# Autodesk Inventor assembly: CCM_Unit_B
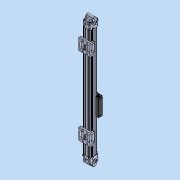
[picture p0: Inventor's stored thumbnail of the model, 180x180]
Saved by Autodesk Inventor 2020 (Build 240168000, 168)
## iProperties
Created: 2021-02-24
Part Number: CCM_Unit_B
Document SubType Name: Assembly
Designer: magnarecta
Author: magnarecta
## Documents named in this file (6)
- C:\Users\lvglv\Documents\GitHub\Eto_Project\Hardware\Parts\CCM\CCM motion linear guide rail\CCM_UNIT\CCM_Unit_B.iam
- C:\Users\lvglv\Documents\GitHub\Eto_Project\Hardware\Parts\CCM\CCM motion linear guide rail\CCM_UNIT\RAIL W40-06.ipt
- C:\Users\lvglv\Documents\GitHub\Eto_Project\Hardware\Parts\CCM\CCM motion linear guide rail\CCM_UNIT\TAILSTOCK W40-00_0+0.ipt
- C:\Users\lvglv\Documents\GitHub\Eto_Project\Hardware\Parts\CCM\CCM motion linear guide rail\CCM_UNIT\CART HK32-06W-00__1.ipt
- C:\Users\lvglv\Documents\GitHub\Eto_Project\Hardware\Parts\CCM\CCM motion linear guide rail\CCM_UNIT\TAILSTOCK W40-00_0+22_1.ipt
- C:\Users\lvglv\Documents\GitHub\Eto_Project\Hardware\Parts\CCM\CCM motion linear guide rail\CCM_UNIT\40 RAIL MOUNT__1.ipt
## Components (6 placed, 5 different names)
1. RAIL W40-06:1 — メイト:2, フラッシュ:3, フラッシュ:4, メイト:3, フラッシュ:5, フラッシュ:6, メイト:6, メイト:7
2. TAILSTOCK W40-00_0+0:1 — メイト:2, フラッシュ:3, フラッシュ:4, メイト:4, メイト:5, メイト:8
3. CART HK32-06W-00__1:1 — メイト:6, メイト:7
4. TAILSTOCK W40-00_0+22_1:1 — メイト:3, フラッシュ:5, フラッシュ:6
5. 40 RAIL MOUNT__1:1 — フラッシュ:7, フラッシュ:8, メイト:4, メイト:5, メイト:8
6. 40 RAIL MOUNT__1:2 — フラッシュ:7, フラッシュ:8
## Relationships (13: Mate 7, Flush 6)
- メイト:2 [Mate]: RAIL W40-06:1 ↔ TAILSTOCK W40-00_0+0:1
- フラッシュ:3 [Flush]: RAIL W40-06:1 ↔ TAILSTOCK W40-00_0+0:1
- フラッシュ:4 [Flush]: RAIL W40-06:1 ↔ TAILSTOCK W40-00_0+0:1
- メイト:3 [Mate]: RAIL W40-06:1 ↔ TAILSTOCK W40-00_0+22_1:1
- フラッシュ:5 [Flush]: RAIL W40-06:1 ↔ TAILSTOCK W40-00_0+22_1:1
- フラッシュ:6 [Flush]: RAIL W40-06:1 ↔ TAILSTOCK W40-00_0+22_1:1
- フラッシュ:7 [Flush]: 40 RAIL MOUNT__1:1 ↔ 40 RAIL MOUNT__1:2
- フラッシュ:8 [Flush]: 40 RAIL MOUNT__1:1 ↔ 40 RAIL MOUNT__1:2
- メイト:4 [Mate]: TAILSTOCK W40-00_0+0:1 ↔ 40 RAIL MOUNT__1:1
- メイト:5 [Mate] (0.05 mm): TAILSTOCK W40-00_0+0:1 ↔ 40 RAIL MOUNT__1:1
- メイト:6 [Mate]: RAIL W40-06:1 ↔ CART HK32-06W-00__1:1
- メイト:7 [Mate]: RAIL W40-06:1 ↔ CART HK32-06W-00__1:1
- メイト:8 [Mate] (50 mm): TAILSTOCK W40-00_0+0:1 ↔ 40 RAIL MOUNT__1:1
